# Autodesk Inventor assembly: MCKL25-5-10
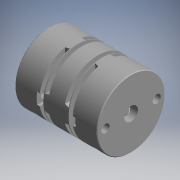
[picture p0: Inventor's stored thumbnail of the model, 180x180]
Saved by Autodesk Inventor 2017.3 (Build 213256000, 256)
## iProperties
Category: PARTsolutions
Company: MISUMI
Part Number: MCKL25-5-10
Catalog Web Link: www.cadenas.de
Description: MCKL, MCKLLK, MCKLRK, MCKLWK-Disc Couplings - High Torque, Set Screw - Double Disc Type
Vendor: MISUMI
Document SubType Name: Assembly
Designer: partserver
Manufacturer: MISUMI
Mass: 10.5735 g
Surface Area: 74.1992 cm^2
Volume: 10.5735 cm^3
Density: 1 g/cm^3
Title: MCKL25-5-10
Author: Cadenas PARTsolutions
Comments: Disc Couplings - High Torque, Set Screw - Double Disc Type
PSOL_IDENT_0: {$CADENAS_DATA\23d-libs\misumi\metric\50_couplings\mckl_asmtab.prj},256 {VTYP=3D},{STYP=ASSTAB},{NB=
PSOL_IDENT_1: MCKL25-5-10},{LINA=MCKL25-5-10},{NN=MCKL, MCKLLK, MCKLRK, MCKLWK},{DATE=30.06.2021 13:24:47},{GEOMDA
PSOL_IDENT_2: TE=08.10.2015 08:23:24},{VERSION=},{LINEID=80},{WBVAR=HS,KGHS,ALT1,DD1,LDC,ALT2,DD2,RDC,ALT3,ALT4},{
PSOL_IDENT_3: WBNUMERIC=DD1,LDC,DD2,RDC}  {NB=MCKL25-5-10},{LINA=MCKL25-5-10},{KT=DUMMY},{PN=MCKL25-5-10},{TYPE=MC
PSOL_IDENT_4: KL},{HS=},{HSALG= '','Standard Hole','KGH','Key Groove Hole' },{KGHS=},{KGHSALG= '','N/A' },{D=25},{
PSOL_IDENT_5: DPN=25},{ALT1=},{ALT1ALG= '','w/o LDC (Shaft Bore Dia. (Left Shaft))','LDC','with LDC (Shaft Bore Di
PSOL_IDENT_6: a. (Left Shaft))' },{DD1=5.00},{DD1ALG=[5,6,6.35,7,8,9.53,10,11,12]},{LDC=0.00},{LDCALG=[0]},{DD1PN=
PSOL_IDENT_7: -5},{DD1LDC=5.000},{ALT2=},{ALT2ALG= '','w/o RDC (Shaft Bore Dia. (Right Shaft))','RDC','with RDC (S
PSOL_IDENT_8: haft Bore Dia. (Right Shaft))' },{DD2=10.00},{DD2ALG=[5,6,6.35,7,8,9.53,10,11,12]},{RDC=0.00},{RDCAL
PSOL_IDENT_9: G=[0]},{DD2PN=-10},{DD2RDC=10.000},{DD3=10.4},{L=30.2},{LL=9.0},{F=4.0},{M=M4},{ALT3=},{ALT3ALG= '','
PSOL_IDENT_10: N/A' },{KLH=0},{BBL=0},{TTL=0.0},{ALT3PN=},{KEYL=0.000},{ALT4=},{ALT4ALG= '','N/A' },{KRH=0},{BBR=0}
PSOL_IDENT_11: ,{TTR=0.0},{ALT4PN=},{KEYR=0.000},{HUBT=4.200},{HUBD=3.000},{HUBL=1.000},{PCD=18.800},{ATAW=9.750},{
PSOL_IDENT_12: ATAH=11.750},{ATAR=12.500},{ATAD=6.688},{ATAT=1.475},{ATADEG=14.000},{DISKD=12.000},{DISKT=0.250},{B
PSOL_IDENT_13: OLTD=3.000},{BOLTH=1.000},{SPCL=5.800},{M3D=4.000},{ML3D=6.000},{LML1=10.000},{LML2=10.000},{RML1=7.
PSOL_IDENT_14: 500},{RML2=7.500},{CP1=2.500},{CP2=2.500},{CP3=5.000},{CP4=5.000},{PPATH=mckl/mckl_asmtpl.prj}
NB: MCKL25-5-10
NN: MCKL, MCKLLK, MCKLRK, MCKLWK
NT: Disc Couplings - High Torque, Set Screw - Double Disc Type
NBSYN: $PN.
LINA: MCKL25-5-10
CATALOG: Misumi
PN: MCKL25-5-10
HS: Standard Hole
KGHS: N/A
D: 25
ALT1: w/o LDC (Shaft Bore Dia. (Left Shaft))
DD1: 5
LDC: 0
ALT2: w/o RDC (Shaft Bore Dia. (Right Shaft))
DD2: 10
RDC: 0
DD3: 10.4
L: 30.2
LL: 9
F: 4
M: M4
ALT3: N/A
KLH: 0
BBL: 0
TTL: 0
ALT4: N/A
KRH: 0
BBR: 0
TTR: 0
SUPPLIER: MISUMI
ARTICLENO: MCKL25-5-10
BOMINFO: MCKL25-5-10
CREATOR: CADENAS GmbH
## Documents named in this file (3)
- e:\temp\worker_3\temp\exporttempdir_908_474_R3CB9\format_0\MCKL25-5-10.iam
- e:\temp\worker_3\temp\exporttempdir_908_474_R3CB9\format_0\MCKL25-5-10_b.ipt
- e:\temp\worker_3\temp\exporttempdir_908_474_R3CB9\format_0\SET-SCREW4-6.ipt
## Components (5 placed, 2 different names)
1. MCKL25-5-10_b:1 — to_set_screw1_Z@1 <-> CP_Z@2, to_set_screw2_Z@1 <-> CP_Z@3, to_set_screw4_Z@1 <-> CP_Z@4, to_set_screw3_Z@1 <-> CP_Z@5
2. SET-SCREW4-6:1 — to_set_screw1_Z@1 <-> CP_Z@2
3. SET-SCREW4-6:2 — to_set_screw2_Z@1 <-> CP_Z@3
4. SET-SCREW4-6:3 — to_set_screw4_Z@1 <-> CP_Z@4
5. SET-SCREW4-6:4 — to_set_screw3_Z@1 <-> CP_Z@5
## Relationships (4: Mate 4)
- to_set_screw1_Z@1 <-> CP_Z@2 [Mate]: MCKL25-5-10_b:1 ↔ SET-SCREW4-6:1
- to_set_screw2_Z@1 <-> CP_Z@3 [Mate]: MCKL25-5-10_b:1 ↔ SET-SCREW4-6:2
- to_set_screw4_Z@1 <-> CP_Z@4 [Mate]: MCKL25-5-10_b:1 ↔ SET-SCREW4-6:3
- to_set_screw3_Z@1 <-> CP_Z@5 [Mate]: MCKL25-5-10_b:1 ↔ SET-SCREW4-6:4
